# Autodesk Inventor assembly: A1-19027 Discharge assembly
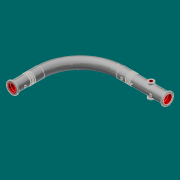
[picture p0: Inventor's stored thumbnail of the model, 180x180]
Saved by Autodesk Inventor 2017.3 (Build 213257000, 257)
## iProperties
Created: 2019-11-15
Part Number: A1-19027 Discharge assembly
Document SubType Name: Assembly
Designer: GVD
Author: GVD
## Documents named in this file (4)
- N:\A1 - Projects\A1-19\A1-19027--Syncrude Aurora HT2 spools - SP-237\A1-19027 Discharge assembly.iam
- N:\A1 - Projects\A1-19\A1-19027--Syncrude Aurora HT2 spools - SP-237\A1-19027-200-00 Spool SP-237-002-P-126-1-A.iam
- N:\A1 - Projects\A1-19\A1-19027--Syncrude Aurora HT2 spools - SP-237\A1-19027-100-00 Spool SP-237-002-P-002-1-B.iam
- N:\A1 - Projects\A1-19\A1-19027--Syncrude Aurora HT2 spools - SP-237\A1-19027-400-00 Spool SP-237-002-P-002-1-C.iam
## Components (3 placed, 3 different names)
1. A1-19027-200-00 Spool SP-237-002-P-126-1-A:1 [sub-assembly] — Insert:1, Angle:1
2. A1-19027-100-00 Spool SP-237-002-P-002-1-B:1 [sub-assembly] — Insert:1, Angle:1, Insert:2, Angle:2
3. A1-19027-400-00 Spool SP-237-002-P-002-1-C:1 [sub-assembly] — Insert:2, Angle:2
## Relationships (4: Insert 2, Angle 2)
- Insert:1 (6 mm): A1-19027-200-00 Spool SP-237-002-P-126-1-A:1 ↔ A1-19027-100-00 Spool SP-237-002-P-002-1-B:1
- Angle:1 (0 deg): A1-19027-200-00 Spool SP-237-002-P-126-1-A:1 ↔ A1-19027-100-00 Spool SP-237-002-P-002-1-B:1
- Insert:2 (1 mm): A1-19027-100-00 Spool SP-237-002-P-002-1-B:1 ↔ A1-19027-400-00 Spool SP-237-002-P-002-1-C:1
- Angle:2 (0 deg): A1-19027-100-00 Spool SP-237-002-P-002-1-B:1 ↔ A1-19027-400-00 Spool SP-237-002-P-002-1-C:1
